# Autodesk Inventor assembly: wafel_rev4
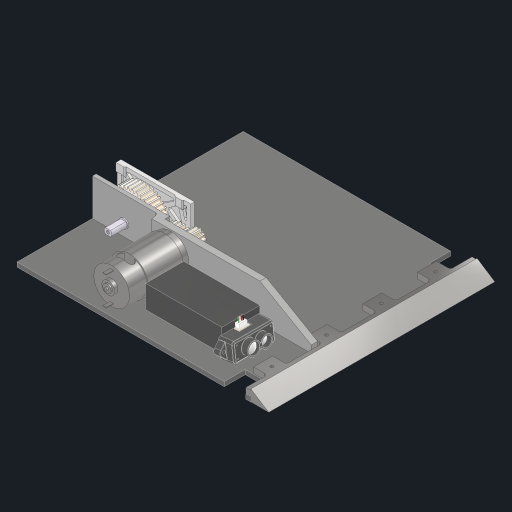
[picture p0: Inventor's stored thumbnail of the model, 512x512]
Saved by Autodesk Inventor 2023 (Build 270158000, 158)
## iProperties
Created: 2024-05-25
Part Number: wafel_rev4
Document SubType Name: Assembly
Designer: szymo
Mass: 531.086 g
Surface Area: 832.687 cm^2
Volume: 163.75 cm^3
Density: 3.24327 g/cm^3
Author: szymo
## iProperties of the stored document TFMINI_S_UART.ipt
Created: 2023-12-04
Part Number: TFMINI S UART
Material: Generic
Description: STEP AP214
Document SubType Name: Modeling
Designer: mateu
Density: 1 g/cm^3
Appearance: Default
Mass: 6.04913 g
Surface Area: 27.6076 cm^2
Volume: 6.04913 cm^3
Sending System: SolidWorks 2016
Preprocessor: SwSTEP 2.0
Title: TFMINI S UART.STEP
Author: USER
Revision Number: ANY
## Documents named in this file (18)
- D:\roboilo\robots\codename wafel - australia\3d_parts\rev4\wafel_rev4.iam
- **D:\roboilo\robots\codename wafel - australia\3d_parts\rev4\wafel_rev4.iam*LocalDocs*xAaaaqfaaAaaaaaaaAaaaqmipQa*TFMINI_S_UART.ipt
- D:\roboilo\robots\codename wafel - australia\3d_parts\rev4\128x32-OLED.ipt
- D:\roboilo\robots\codename wafel - australia\3d_parts\rev4\interface_board.ipt
- D:\roboilo\robots\codename wafel - australia\3d_parts\rev4\KTIR-Board.ipt
- D:\roboilo\robots\codename wafel - australia\3d_parts\rev4\motor_w_gear.iam
- D:\roboilo\robots\codename wafel - australia\3d_parts\rev4\plog.ipt
- D:\roboilo\robots\codename wafel - australia\3d_parts\rev4\smolgear_shaft.ipt
- D:\roboilo\robots\codename wafel - australia\3d_parts\rev4\stack.iam
- D:\roboilo\robots\codename wafel - australia\3d_parts\rev4\Switch.ipt
- D:\roboilo\robots\codename wafel - australia\3d_parts\rev4\wheel_axle.iam
- D:\roboilo\robots\codename wafel - australia\3d_parts\rev4\Design Accelerator\smolGear.iam
- D:\roboilo\robots\codename wafel - australia\3d_parts\rev4\lipo3s650mah.ipt
- D:\roboilo\robots\codename wafel - australia\3d_parts\rev4\lipo2s450mah.ipt
- D:\roboilo\robots\codename wafel - australia\3d_parts\rev4\base.ipt
- D:\roboilo\robots\codename wafel - australia\3d_parts\rev4\side_r.ipt
- D:\roboilo\robots\codename wafel - australia\3d_parts\rev4\r_gaerHold.ipt
- D:\roboilo\robots\codename wafel - australia\3d_parts\rev4\TFMINI_S_UART.ipt
## Components (23 placed, 16 different names)
1. base:1 — Mate:3, Mate:4, Flush:5, Tangent:1, Tangent:2, Angle:2, Tangent:8, Tangent:10, Mate:5, Mate:6, Mate:9, Mate:10, Mate:12, Mate:13, Angle:6, Mate:14, Mate:15, Tangent:11, Tangent:12, Tangent:13, Tangent:14, Flush:18
2. plog:1 — Mate:3, Mate:4, Flush:5, Flush:10, Angle:1, Angle:3, Angle:4, Flush:11, Mate:11, Angle:5, Angle:7, Angle:8, Mate:16, Mate:17
3. side_r:1 — Flush:14, Flush:16
4. r_gaerHold:1 — Mate:18, Flush:18
5. stack:1 [sub-assembly] — Flush:10, Mate:5, Mate:7, Mate:8, Mate:11
6. motor_w_gear:1 [sub-assembly] — Tangent:1, Angle:2, Flush:8, Flush:9, Tangent:3, Mate:7, Tangent:11, Flush:14, Flush:16
7. wheel_axle:1 [sub-assembly] — Flush:9, Tangent:4, Tangent:10, Angle:3, Mate:10, Mate:18
8. smolGear:1 [sub-assembly] — Mate:1, Flush:8, Tangent:3, Tangent:4, Flush:13
9. smolgear_shaft:1 — Mate:1, Flush:13, Tangent:14
10. motor_w_gear:2 [sub-assembly] — Tangent:2, Angle:1, Flush:6, Flush:7, Tangent:5, Mate:8, Tangent:12
11. wheel_axle:2 [sub-assembly] — Flush:7, Tangent:6, Tangent:8, Angle:4, Mate:9
12. smolGear:2 [sub-assembly] — Mate:2, Flush:6, Tangent:5, Tangent:6, Flush:12
13. smolgear_shaft:2 — Mate:2, Flush:12, Tangent:13
14. lipo3s650mah:1 — Mate:15
15. lipo2s450mah:1 — Flush:11, Mate:6
16. lipo3s650mah:2 — Mate:14
17. TFMINI_S_UART:2 — Mate:12, Angle:5, Angle:7, Mate:17
18. TFMINI_S_UART:1 — Mate:13, Angle:6, Angle:8, Mate:16
19. KTIR-Board:1
20. KTIR-Board:2
21. 128x32-OLED:1
22. interface_board:1
23. Switch:1
## Relationships (50: Mate 18, Flush 12, Tangent 12, Angle 8)
- Mate:1: smolGear:1 ↔ smolgear_shaft:1
- Mate:2: smolGear:2 ↔ smolgear_shaft:2
- Mate:3: base:1 ↔ plog:1
- Mate:4: base:1 ↔ plog:1
- Flush:5: base:1 ↔ plog:1
- Tangent:1: base:1 ↔ motor_w_gear:1
- Tangent:2: base:1 ↔ motor_w_gear:2
- Angle:1 (0 deg): plog:1 ↔ motor_w_gear:2
- Angle:2 (0 deg): base:1 ↔ motor_w_gear:1
- Flush:6: motor_w_gear:2 ↔ smolGear:2
- Flush:7: motor_w_gear:2 ↔ wheel_axle:2
- Flush:8: motor_w_gear:1 ↔ smolGear:1
- Flush:9: motor_w_gear:1 ↔ wheel_axle:1
- Tangent:3: motor_w_gear:1 ↔ smolGear:1
- Tangent:4: wheel_axle:1 ↔ smolGear:1
- Tangent:5: motor_w_gear:2 ↔ smolGear:2
- Tangent:6: wheel_axle:2 ↔ smolGear:2
- Tangent:8 (4 mm): base:1 ↔ wheel_axle:2
- Tangent:10 (4 mm): base:1 ↔ wheel_axle:1
- Flush:10 (61.5 mm): plog:1 ↔ stack:1
- Mate:5 (2 mm): base:1 ↔ stack:1
- Angle:3 (0 deg): plog:1 ↔ wheel_axle:1
- Angle:4 (0 deg): plog:1 ↔ wheel_axle:2
- Flush:11 (82 mm): plog:1 ↔ lipo2s450mah:1
- Mate:6: base:1 ↔ lipo2s450mah:1
- Flush:12 (2 mm): smolGear:2 ↔ smolgear_shaft:2
- Flush:13 (-2 mm): smolGear:1 ↔ smolgear_shaft:1
- Mate:7 (8 mm): stack:1 ↔ motor_w_gear:1
- Mate:8 (8 mm): stack:1 ↔ motor_w_gear:2
- Mate:9 (-25 mm): base:1 ↔ wheel_axle:2
- Mate:10 (-25 mm): base:1 ↔ wheel_axle:1
- Mate:11 (10 mm): plog:1 ↔ stack:1
- Mate:12: base:1 ↔ TFMINI_S_UART:2
- Angle:5 (-7 deg): plog:1 ↔ TFMINI_S_UART:2
- Mate:13: base:1 ↔ TFMINI_S_UART:1
- Angle:6 (-7 deg): base:1 ↔ TFMINI_S_UART:1
- Angle:7 (180 deg): plog:1 ↔ TFMINI_S_UART:2
- Angle:8 (180 deg): plog:1 ↔ TFMINI_S_UART:1
- Mate:14: base:1 ↔ lipo3s650mah:2
- Mate:15: base:1 ↔ lipo3s650mah:1
- Tangent:11 (52.5 mm): base:1 ↔ motor_w_gear:1
- Tangent:12 (52.5 mm): base:1 ↔ motor_w_gear:2
- Tangent:13 (2.55 mm): base:1 ↔ smolgear_shaft:2
- Tangent:14 (2.55 mm): base:1 ↔ smolgear_shaft:1
- Mate:16 (22 mm): plog:1 ↔ TFMINI_S_UART:1
- Mate:17 (22 mm): plog:1 ↔ TFMINI_S_UART:2
- Flush:14: side_r:1 ↔ motor_w_gear:1
- Flush:16: side_r:1 ↔ motor_w_gear:1
- Mate:18: r_gaerHold:1 ↔ wheel_axle:1
- Flush:18: base:1 ↔ r_gaerHold:1
